# Autodesk Inventor assembly: Shooter
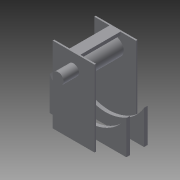
[picture p0: Inventor's stored thumbnail of the model, 180x180]
Saved by Autodesk Inventor 2014 (Build 180170000, 170)
## iProperties
Created: 2016-01-22
Part Number: Shooter
Document SubType Name: Assembly
Designer: shawnsargent
Author: shawnsargent
## Documents named in this file (4)
- Z:\Robot\Shooter.iam
- Z:\Robot\Robotics ball launcher guide.ipt
- Z:\Robot\Robotics ball launcher motor frame.ipt
- C:\Users\shawnsargent\Documents\Base.ipt
## Components (3 placed, 3 different names)
1. Robotics ball launcher guide:1 — Flush:1, Mate:1, Flush:2, Flush:3, Mate:2
2. Robotics ball launcher motor frame:1 — Flush:1, Mate:1, Flush:2, Flush:4
3. Base:1 — Flush:3, Flush:4, Mate:2
## Relationships (6: Flush 4, Mate 2)
- Flush:1: Robotics ball launcher guide:1 ↔ Robotics ball launcher motor frame:1
- Mate:1 (59.7408 mm): Robotics ball launcher guide:1 ↔ Robotics ball launcher motor frame:1
- Flush:2 (-116.1313 mm): Robotics ball launcher guide:1 ↔ Robotics ball launcher motor frame:1
- Flush:3: Robotics ball launcher guide:1 ↔ Base:1
- Flush:4: Robotics ball launcher motor frame:1 ↔ Base:1
- Mate:2: Robotics ball launcher guide:1 ↔ Base:1
